# Autodesk Inventor assembly: inner
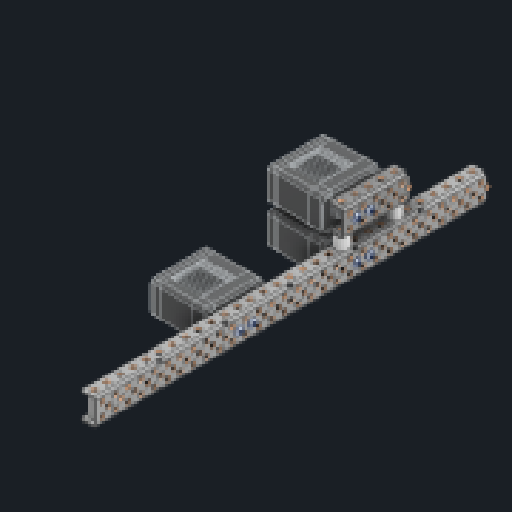
[picture p0: Inventor's stored thumbnail of the model, 512x512]
Saved by Autodesk Inventor 2025 (Build 290162000, 162)
## iProperties
Created: 2024-10-03
Part Number: inner
Document SubType Name: Assembly
Designer: Averey Ku
Author: Averey Ku
## Documents named in this file (9)
- D:\vex_robotics_high_stakes\hardware\cad\bots\high_stakes_v2\chassis\drivebay\inner.iam
- D:\vex_robotics_high_stakes\hardware\cad\robpros_cad_lib\Structure\C Channel\Aluminum 1x2x1\Alu C 1x2x1x30.ipt
- D:\vex_robotics_high_stakes\hardware\cad\robpros_cad_lib\Motion\Spacers\Spacer Nylon .500 OD\NSpacer White .500 OD x .500.ipt
- D:\vex_robotics_high_stakes\hardware\cad\robpros_cad_lib\Motion\Spacers\Spacer Nylon .500 OD.ipt
- D:\vex_robotics_high_stakes\hardware\cad\robpros_cad_lib\Structure\C Channel\Aluminum 1x2x1\Alu C 1x2x1x5.ipt
- D:\vex_robotics_high_stakes\hardware\cad\robpros_cad_lib\Electronics\Motors with Screws\SteelM-StarS.iam
- D:\vex_robotics_high_stakes\hardware\cad\robpros_cad_lib\Electronics\Motors with Screws.iam
- D:\vex_robotics_high_stakes\hardware\cad\VEX-CAD-Inventor\Structure\Standoff\Standoff .875.ipt
- D:\vex_robotics_high_stakes\hardware\cad\VEX-CAD-Inventor\Structure\Standoff.ipt
## Components (9 placed, 5 different names)
1. Alu C 1x2x1x30:1 — Mate:2, Insert:5, Insert:6, Mate:4, Insert:7, Insert:8
2. NSpacer White .500 OD x .500:1
3. NSpacer White .500 OD x .500:2
4. Alu C 1x2x1x5:1 — Insert:4, Mate:3
5. SteelM-StarS:1 [sub-assembly] — Insert:4, Mate:3
6. SteelM-StarS:2 [sub-assembly] — Insert:6, Mate:4
7. SteelM-StarS:3 [sub-assembly] — Insert:5
8. Standoff .875:1 — Insert:7
9. Standoff .875:2 — Insert:8
## Relationships (12: Insert 8, Mate 4)
- [Insert]: Alu C 1x2x1x30:1 ↔ NSpacer White .500 OD x .500:2
- [Insert]: Alu C 1x2x1x30:1 ↔ NSpacer White .500 OD x .500:1
- [Insert]: NSpacer White .500 OD x .500:1 ↔ Alu C 1x2x1x5:1
- [Mate]: NSpacer White .500 OD x .500:2 ↔ Alu C 1x2x1x5:1
- Mate:2: Alu C 1x2x1x30:1
- Insert:4: Alu C 1x2x1x5:1 ↔ SteelM-StarS:1
- Mate:3: Alu C 1x2x1x5:1 ↔ SteelM-StarS:1
- Insert:5: Alu C 1x2x1x30:1 ↔ SteelM-StarS:3
- Insert:6: Alu C 1x2x1x30:1 ↔ SteelM-StarS:2
- Mate:4: Alu C 1x2x1x30:1 ↔ SteelM-StarS:2
- Insert:7: Alu C 1x2x1x30:1 ↔ Standoff .875:1
- Insert:8: Alu C 1x2x1x30:1 ↔ Standoff .875:2
